# Autodesk Inventor assembly: Assembly1
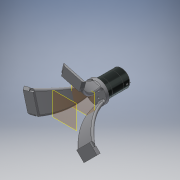
[picture p0: Inventor's stored thumbnail of the model, 180x180]
Saved by Autodesk Inventor 2019.4 (Build 234330000, 330)
## iProperties
Created: 2019-10-16
Part Number: Assembly1
Document SubType Name: Assembly
Designer: Jorian Bruslind
Author: Jorian Bruslind
## Documents named in this file (3)
- C:\Users\Jorian Bruslind\Documents\GitHub\PersonalProjects\Underwater Parts\Ebay_Motor\Assembly1.iam
- C:\Users\Jorian Bruslind\Documents\GitHub\PersonalProjects\Underwater Parts\Ebay_Motor\Motor.ipt
- C:\Users\Jorian Bruslind\Documents\GitHub\PersonalProjects\Underwater Parts\Ebay_Motor\Motor_Testmount.ipt
## Components (2 placed, 2 different names)
1. Motor:1 — Mate:1, Mate:2, Mate:3
2. Motor_Testmount:1 — Mate:1, Mate:2, Mate:3
## Relationships (3: Mate 3)
- Mate:1: Motor:1 ↔ Motor_Testmount:1
- Mate:2: Motor:1 ↔ Motor_Testmount:1
- Mate:3: Motor:1 ↔ Motor_Testmount:1
